# Autodesk Inventor assembly: FE-00035
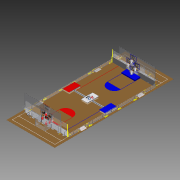
[picture p0: Inventor's stored thumbnail of the model, 180x180]
Saved by Autodesk Inventor 2012 (Build 160160000, 160)
## iProperties
Created: 2011-05-23
Part Number: FE-00035
Document SubType Name: Assembly
Designer: dfoster
Author: dfoster
## Documents named in this file (11)
- C:\Data Folder\FRC 2012 Field\FRC 2012 Competition Field.iam
- C:\Data Folder\FRC 2012 Field\Components\FE-00035-06.ipt
- C:\Data Folder\FRC 2012 Field\Components\FE-00035-02.iam
- C:\Data Folder\FRC 2012 Field\Components\FE-00035-01.iam
- C:\Data Folder\FRC 2012 Field\Components\GE-12017.iam
- C:\Data Folder\FRC 2012 Field\Components\Tape_lane.ipt
- C:\Data Folder\FRC 2012 Field\Components\GE-12058.ipt
- C:\Data Folder\FRC 2012 Field\Components\GE-12050.ipt
- C:\Data Folder\FRC 2012 Field\Components\Tape_key.ipt
- C:\Data Folder\FRC 2012 Field\Components\FE-00035-05.ipt
- C:\Data Folder\FRC 2012 Field\Components\logo.ipt
## Components (21 placed, 10 different names)
1. FE-00035-06:1 — Flush:2, Flush:3, Flush:4, Mate:1, Mate:29, Mate:31, Mate:33, Mate:60, Mate:61, Mate:65, Mate:67, Mate:69, Mate:71, Mate:72, Mate:75, Mate:76, Mate:80, Mate:81, Mate:84, Mate:87, Mate:90, Mate:92
2. FE-00035-02:1 [sub-assembly] — Flush:1, Mate:1, Mate:28, Mate:30, Mate:62, Mate:78, Mate:91, Flush:39
3. FE-00035-02:2 [sub-assembly] — Mate:33, Mate:34, Mate:35, Mate:63, Mate:83, Mate:93, Flush:40
4. FE-00035-01:1 [sub-assembly] — Mate:28, Mate:29, Mate:35, Mate:36, Flush:27
5. FE-00035-01:2 [sub-assembly] — Mate:30, Mate:31, Mate:34, Flush:26
6. GE-12017:1 [sub-assembly] — Mate:65, Mate:66, Flush:29, Mate:68, Flush:30, Mate:73, Flush:31, Mate:94, Flush:41, Flush:42
7. GE-12058:1 — Mate:72, Mate:73, Flush:31, Flush:32, Mate:74
8. GE-12058:2 — Mate:67, Flush:29, Mate:68, Mate:70
9. Tape_lane:1 — Mate:61, Mate:62, Flush:27
10. Tape_lane:2 — Mate:60, Mate:63, Flush:26
11. GE-12017:2 [sub-assembly] — Mate:71, Flush:32, Mate:74
12. GE-12017:3 [sub-assembly] — Mate:69, Flush:30, Mate:70
13. GE-12050:1 — Mate:75, Mate:77, Flush:36, Mate:78, Mate:79, Flush:38, Mate:85, Mate:86
14. GE-12050:2 — Mate:76, Mate:77, Flush:36
15. GE-12050:3 — Mate:80, Mate:82, Flush:37, Mate:83
16. GE-12050:4 — Mate:81, Mate:82, Flush:37, Flush:38, Mate:88, Mate:89
17. Tape_key:1 — Mate:84, Mate:85, Mate:86
18. Tape_key:2 — Mate:87, Mate:88, Mate:89
19. FE-00035-05:1 — Mate:90, Mate:91, Flush:39
20. FE-00035-05:2 — Mate:92, Mate:93, Flush:40
21. logo:1 — Mate:94, Flush:41, Flush:42
## Relationships (63: Mate 45, Flush 18)
- Flush:1: FE-00035-02:1
- Flush:2: FE-00035-06:1
- Flush:3: FE-00035-06:1
- Flush:4: FE-00035-06:1
- Mate:1: FE-00035-06:1 ↔ FE-00035-02:1
- Mate:28: FE-00035-02:1 ↔ FE-00035-01:1
- Mate:29: FE-00035-06:1 ↔ FE-00035-01:1
- Mate:30: FE-00035-02:1 ↔ FE-00035-01:2
- Mate:31: FE-00035-06:1 ↔ FE-00035-01:2
- Mate:33: FE-00035-06:1 ↔ FE-00035-02:2
- Mate:34: FE-00035-02:2 ↔ FE-00035-01:2
- Mate:35: FE-00035-02:2 ↔ FE-00035-01:1
- Mate:36: FE-00035-01:1
- [Mate]: FE-00035-06:1 ↔ GE-12058:1
- [Mate]: FE-00035-06:1 ↔ GE-12058:2
- Mate:60: FE-00035-06:1 ↔ Tape_lane:2
- Mate:61: FE-00035-06:1 ↔ Tape_lane:1
- Mate:62: FE-00035-02:1 ↔ Tape_lane:1
- Mate:63: FE-00035-02:2 ↔ Tape_lane:2
- Flush:26 (-1295.4 mm): FE-00035-01:2 ↔ Tape_lane:2
- Flush:27 (-1295.4 mm): FE-00035-01:1 ↔ Tape_lane:1
- [Flush]: GE-12017:1
- Mate:65: FE-00035-06:1 ↔ GE-12017:1
- Mate:66: GE-12017:1
- Mate:67: FE-00035-06:1 ↔ GE-12058:2
- Flush:29: GE-12017:1 ↔ GE-12058:2
- Mate:68 (3.175 mm): GE-12017:1 ↔ GE-12058:2
- Mate:69: FE-00035-06:1 ↔ GE-12017:3
- Flush:30: GE-12017:1 ↔ GE-12017:3
- Mate:70 (3.175 mm): GE-12058:2 ↔ GE-12017:3
- Mate:71: FE-00035-06:1 ↔ GE-12017:2
- Mate:72: FE-00035-06:1 ↔ GE-12058:1
- Mate:73 (3.175 mm): GE-12017:1 ↔ GE-12058:1
- Flush:31: GE-12017:1 ↔ GE-12058:1
- Flush:32: GE-12058:1 ↔ GE-12017:2
- Mate:74 (3.175 mm): GE-12058:1 ↔ GE-12017:2
- Mate:75: FE-00035-06:1 ↔ GE-12050:1
- Mate:76: FE-00035-06:1 ↔ GE-12050:2
- Mate:77: GE-12050:1 ↔ GE-12050:2
- Flush:36: GE-12050:1 ↔ GE-12050:2
- Mate:78 (3657.6 mm): FE-00035-02:1 ↔ GE-12050:1
- Mate:79: GE-12050:1
- Mate:80: FE-00035-06:1 ↔ GE-12050:3
- Mate:81: FE-00035-06:1 ↔ GE-12050:4
- Mate:82: GE-12050:3 ↔ GE-12050:4
- Flush:37: GE-12050:3 ↔ GE-12050:4
- Flush:38: GE-12050:1 ↔ GE-12050:4
- Mate:83 (3657.6 mm): FE-00035-02:2 ↔ GE-12050:3
- Mate:84: FE-00035-06:1 ↔ Tape_key:1
- Mate:85: GE-12050:1 ↔ Tape_key:1
- Mate:86: GE-12050:1 ↔ Tape_key:1
- Mate:87: FE-00035-06:1 ↔ Tape_key:2
- Mate:88: GE-12050:4 ↔ Tape_key:2
- Mate:89: GE-12050:4 ↔ Tape_key:2
- Mate:90: FE-00035-06:1 ↔ FE-00035-05:1
- Mate:91: FE-00035-02:1 ↔ FE-00035-05:1
- Flush:39: FE-00035-02:1 ↔ FE-00035-05:1
- Mate:92: FE-00035-06:1 ↔ FE-00035-05:2
- Mate:93: FE-00035-02:2 ↔ FE-00035-05:2
- Flush:40: FE-00035-02:2 ↔ FE-00035-05:2
- Mate:94 (-6.35 mm): GE-12017:1 ↔ logo:1
- Flush:41: GE-12017:1 ↔ logo:1
- Flush:42 (508 mm): GE-12017:1 ↔ logo:1
